# Autodesk Inventor assembly: A2017_T4_04
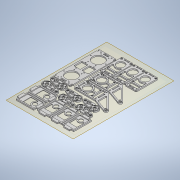
[picture p0: Inventor's stored thumbnail of the model, 180x180]
Saved by Autodesk Inventor 2020 (Build 240168000, 168)
## iProperties
Created: 2021-08-27
Part Number: A2017_T4_04
Document SubType Name: Assembly
Designer: Masato
Author: Masato
## Documents named in this file (7)
- C:\Users\naoki\Documents\Inventor\CitBrains\git_clone\SUSTAINA_ver1_0\AT4_173\SUSTAINA-OP\Cam\A2017_T4_04.iam
- C:\Users\naoki\Documents\Inventor\CitBrains\git_clone\SUSTAINA_ver1_0\AT4_173\SUSTAINA-OP\Cam\DisposableBoard.ipt
- C:\Users\naoki\Documents\Inventor\CitBrains\git_clone\SUSTAINA_ver1_0\AT4_173\SUSTAINA-OP\UpperBody\Trunk\Trunk_servo_bottom_frame.ipt
- C:\Users\naoki\Documents\Inventor\CitBrains\git_clone\SUSTAINA_ver1_0\AT4_173\SUSTAINA-OP\LowerBody\Ankle\Ankle_side_pitch_frame.ipt
- C:\Users\naoki\Documents\Inventor\CitBrains\git_clone\SUSTAINA_ver1_0\AT4_173\SUSTAINA-OP\UpperBody\Trunk\Trunk_waisit_frame.ipt
- C:\Users\naoki\Documents\Inventor\CitBrains\git_clone\SUSTAINA_ver1_0\AT4_173\SUSTAINA-OP\UpperBody\Trunk\Trunk_shoulder_frame_MIR.ipt
- C:\Users\naoki\Documents\Inventor\CitBrains\git_clone\SUSTAINA_ver1_0\AT4_173\SUSTAINA-OP\UpperBody\Trunk\Trunk_neck_frame.ipt
## Components (18 placed, 6 different names)
1. DisposableBoard:1 — メイト:2, メイト:1, フラッシュ:1, フラッシュ:2, メイト:4, メイト:5, メイト:6, メイト:7, メイト:9, フラッシュ:3, フラッシュ:4, メイト:17, メイト:18, メイト:19, メイト:20, 正接:1, メイト:28, メイト:29, 正接:6, メイト:32, メイト:34, メイト:35, フラッシュ:10, メイト:40
2. Trunk_servo_bottom_frame:1 — メイト:4, メイト:11, フラッシュ:6, メイト:21, 正接:2
3. Trunk_servo_bottom_frame:2 — メイト:6, フラッシュ:8, フラッシュ:9, メイト:12, メイト:13
4. Trunk_servo_bottom_frame:3 — メイト:7, フラッシュ:3, フラッシュ:4, メイト:11, フラッシュ:6, フラッシュ:7, メイト:14
5. Trunk_servo_bottom_frame:4 — メイト:5, フラッシュ:7, フラッシュ:8, メイト:13, メイト:14, メイト:24
6. Trunk_servo_bottom_frame:6 — メイト:9, フラッシュ:9, メイト:12, メイト:31, 正接:7
7. Ankle_side_pitch_frame:1 — メイト:17, メイト:22, 正接:3, 正接:6, メイト:37
8. Ankle_side_pitch_frame:2 — メイト:18, メイト:21, 正接:1, メイト:22
9. Ankle_side_pitch_frame:3 — メイト:20, メイト:24, 正接:2, メイト:25, 正接:4
10. Ankle_side_pitch_frame:4 — メイト:19, メイト:25, 正接:3, 正接:5
11. Ankle_side_pitch_frame:5 — メイト:28, メイト:30, メイト:31, 正接:4
12. Ankle_side_pitch_frame:6 — メイト:29, メイト:30, 正接:5, 正接:8
13. Trunk_waisit_frame:1 — メイト:34, フラッシュ:10, メイト:37, メイト:39
14. Trunk_shoulder_frame_MIR:1 — メイト:32, メイト:36, 正接:7, 正接:8, フラッシュ:11
15. Trunk_shoulder_frame_MIR:2 — メイト:35, メイト:36, フラッシュ:11, メイト:38
16. Trunk_neck_frame:1 — メイト:38, メイト:39, メイト:40
17. Trunk_neck_frame:2
18. Trunk_neck_frame:3
## Component patterns: (3 elements, first: Trunk_neck_frame:1)
## Relationships (49: Mate 31, Flush 10, Tangent 8)
- メイト:2 [Mate]: DisposableBoard:1
- メイト:1 [Mate]: DisposableBoard:1
- フラッシュ:1 [Flush]: DisposableBoard:1
- フラッシュ:2 [Flush]: DisposableBoard:1
- メイト:4 [Mate]: DisposableBoard:1 ↔ Trunk_servo_bottom_frame:1
- メイト:5 [Mate]: DisposableBoard:1 ↔ Trunk_servo_bottom_frame:4
- メイト:6 [Mate]: DisposableBoard:1 ↔ Trunk_servo_bottom_frame:2
- メイト:7 [Mate]: DisposableBoard:1 ↔ Trunk_servo_bottom_frame:3
- メイト:9 [Mate]: DisposableBoard:1 ↔ Trunk_servo_bottom_frame:6
- フラッシュ:3 [Flush] (1.5 mm): DisposableBoard:1 ↔ Trunk_servo_bottom_frame:3
- フラッシュ:4 [Flush] (1.5 mm): DisposableBoard:1 ↔ Trunk_servo_bottom_frame:3
- メイト:11 [Mate] (2.5 mm): Trunk_servo_bottom_frame:1 ↔ Trunk_servo_bottom_frame:3
- フラッシュ:6 [Flush]: Trunk_servo_bottom_frame:1 ↔ Trunk_servo_bottom_frame:3
- フラッシュ:7 [Flush]: Trunk_servo_bottom_frame:3 ↔ Trunk_servo_bottom_frame:4
- フラッシュ:8 [Flush]: Trunk_servo_bottom_frame:2 ↔ Trunk_servo_bottom_frame:4
- フラッシュ:9 [Flush]: Trunk_servo_bottom_frame:2 ↔ Trunk_servo_bottom_frame:6
- メイト:12 [Mate] (2.5 mm): Trunk_servo_bottom_frame:2 ↔ Trunk_servo_bottom_frame:6
- メイト:13 [Mate] (2.5 mm): Trunk_servo_bottom_frame:2 ↔ Trunk_servo_bottom_frame:4
- メイト:14 [Mate] (2.5 mm): Trunk_servo_bottom_frame:3 ↔ Trunk_servo_bottom_frame:4
- メイト:17 [Mate]: DisposableBoard:1 ↔ Ankle_side_pitch_frame:1
- メイト:18 [Mate]: DisposableBoard:1 ↔ Ankle_side_pitch_frame:2
- メイト:19 [Mate]: DisposableBoard:1 ↔ Ankle_side_pitch_frame:4
- メイト:20 [Mate]: DisposableBoard:1 ↔ Ankle_side_pitch_frame:3
- メイト:21 [Mate] (2.5 mm): Trunk_servo_bottom_frame:1 ↔ Ankle_side_pitch_frame:2
- 正接:1 [Tangent] (1.5 mm): DisposableBoard:1 ↔ Ankle_side_pitch_frame:2
- メイト:22 [Mate] (2.5 mm): Ankle_side_pitch_frame:1 ↔ Ankle_side_pitch_frame:2
- メイト:24 [Mate] (2.5 mm): Trunk_servo_bottom_frame:4 ↔ Ankle_side_pitch_frame:3
- 正接:2 [Tangent] (2.5 mm): Trunk_servo_bottom_frame:1 ↔ Ankle_side_pitch_frame:3
- メイト:25 [Mate] (2.5 mm): Ankle_side_pitch_frame:3 ↔ Ankle_side_pitch_frame:4
- 正接:3 [Tangent] (2.5 mm): Ankle_side_pitch_frame:1 ↔ Ankle_side_pitch_frame:4
- メイト:28 [Mate]: DisposableBoard:1 ↔ Ankle_side_pitch_frame:5
- メイト:29 [Mate]: DisposableBoard:1 ↔ Ankle_side_pitch_frame:6
- メイト:30 [Mate] (2.5 mm): Ankle_side_pitch_frame:5 ↔ Ankle_side_pitch_frame:6
- メイト:31 [Mate] (2.5 mm): Trunk_servo_bottom_frame:6 ↔ Ankle_side_pitch_frame:5
- 正接:4 [Tangent] (2.5 mm): Ankle_side_pitch_frame:3 ↔ Ankle_side_pitch_frame:5
- 正接:5 [Tangent] (2.5 mm): Ankle_side_pitch_frame:4 ↔ Ankle_side_pitch_frame:6
- 正接:6 [Tangent] (2.5 mm): DisposableBoard:1 ↔ Ankle_side_pitch_frame:1
- メイト:32 [Mate]: DisposableBoard:1 ↔ Trunk_shoulder_frame_MIR:1
- メイト:34 [Mate]: DisposableBoard:1 ↔ Trunk_waisit_frame:1
- メイト:35 [Mate]: DisposableBoard:1 ↔ Trunk_shoulder_frame_MIR:2
- メイト:36 [Mate] (2.5 mm): Trunk_shoulder_frame_MIR:1 ↔ Trunk_shoulder_frame_MIR:2
- 正接:7 [Tangent]: Trunk_servo_bottom_frame:6 ↔ Trunk_shoulder_frame_MIR:1
- 正接:8 [Tangent] (2.5 mm): Ankle_side_pitch_frame:6 ↔ Trunk_shoulder_frame_MIR:1
- フラッシュ:10 [Flush] (2 mm): DisposableBoard:1 ↔ Trunk_waisit_frame:1
- メイト:37 [Mate] (2.5 mm): Ankle_side_pitch_frame:1 ↔ Trunk_waisit_frame:1
- フラッシュ:11 [Flush]: Trunk_shoulder_frame_MIR:1 ↔ Trunk_shoulder_frame_MIR:2
- メイト:38 [Mate] (2.5 mm): Trunk_shoulder_frame_MIR:2 ↔ Trunk_neck_frame:1
- メイト:39 [Mate] (2.5 mm): Trunk_waisit_frame:1 ↔ Trunk_neck_frame:1
- メイト:40 [Mate]: DisposableBoard:1 ↔ Trunk_neck_frame:1
